# Autodesk Inventor assembly: assembly
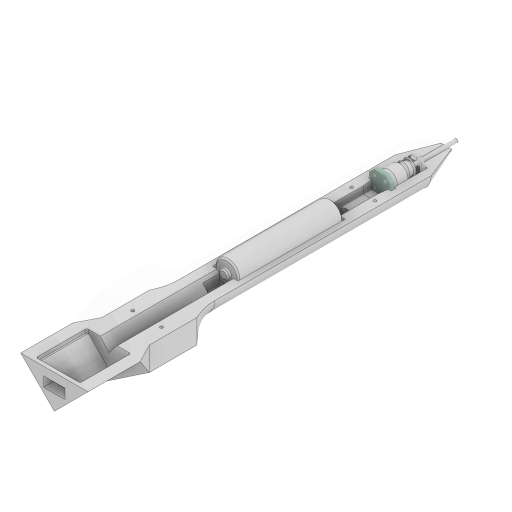
[picture p0: Inventor's stored thumbnail of the model, 512x512]
Saved by Autodesk Inventor 2023 (Build 270158000, 158)
## iProperties
Created: 2023-03-22
Part Number: assembly
Document SubType Name: Assembly
Designer: James
Author: James
## iProperties of the stored document dpoint PCB.ipt
Created: 2023-07-01
Part Number: dpoint PCB
Material: Generic
Document SubType Name: Modeling
Designer: James
Density: 1 g/cm^3
Appearance: Default
Author: James
## iProperties of the stored document COMPOUND.ipt
Created: 2023-07-01
Part Number: COMPOUND
Material: Generic
Document SubType Name: Modeling
Designer: James
Density: 1 g/cm^3
Appearance: Default
Author: James
## iProperties of the stored document ForceSensor(HSFPAR003A).iam
Created: 2023-07-01
Part Number: ForceSensor(HSFPAR003A)
Document SubType Name: Assembly
Designer: James
Author: James
## iProperties of the stored document dpoint.iam
Company: Kicad
Created: 2023-07-02
Part Number: dpoint 1
Description: KiCad electronic assembly
Document SubType Name: Assembly
Designer: James
Authority: Unknown
Sending System: KiCad to STEP converter
Preprocessor: Open CASCADE STEP processor 7.6
Title: dpoint.step
Author: Pcbnew
## Documents named in this file (12)
- C:\Users\James\OneDrive\Documents\Uni\2023_S1\ENG401_honours\inventor\assembly.iam
- C:\Users\James\OneDrive\Documents\Uni\2023_S1\ENG401_honours\inventor\stlyus_body.ipt
- C:\Users\James\OneDrive\Documents\Uni\2023_S1\ENG401_honours\inventor\stylus_nib.ipt
- C:\Users\James\OneDrive\Documents\Uni\2023_S1\ENG401_honours\inventor\seed_arduino.ipt
- C:\Users\James\OneDrive\Documents\Uni\2023_S1\ENG401_honours\inventor\stylus_nib_base.ipt
- C:\Users\James\OneDrive\Documents\Uni\2023_S1\ENG401_honours\inventor\Compress Spring11.ipt
- **C:\Users\James\OneDrive\Documents\Uni\2023_S1\ENG401_honours\inventor\assembly.iam*LocalDocs*xAaaaqsaaAaaaaaaaAaaaqwdiHg*dpoint.iam
- C:\Users\James\OneDrive\Documents\Uni\2023_S1\ENG401_honours\inventor\batt_10440.ipt
- **C:\Users\James\OneDrive\Documents\Uni\2023_S1\ENG401_honours\inventor\assembly.iam*LocalDocs*xAaaaq4daAaaaaaaaAaaaqsjtPd*dpoint PCB.ipt
- **C:\Users\James\OneDrive\Documents\Uni\2023_S1\ENG401_honours\inventor\assembly.iam*LocalDocs*xAaaaavbaAaaaaaaaAaaaaf43Ph*COMPOUND.ipt
- **C:\Users\James\OneDrive\Documents\Uni\2023_S1\ENG401_honours\inventor\assembly.iam*LocalDocs*xAaaaqdbaAaaaaaaaAaaaqo3uAf*ForceSensor(HSFPAR003A).iam
- C:\Users\James\OneDrive\Documents\Uni\2023_S1\ENG401_honours\inventor\dpoint.step
## Components (8 placed, 7 different names)
1. stlyus_body:1 — Mate:1, Flush:1, Mate:2, Mate:3, Flush:2, Flush:7, Flush:3, Mate:8, Mate:9, Insert:2
2. stlyus_body:2 — Mate:1, Flush:1, Mate:2, Mate:7, Flush:8
3. stylus_nib:1 — Mate:3, Insert:1
4. seed_arduino:1 — Flush:2, Flush:7, Flush:3
5. stylus_nib_base:1 — Insert:1, Mate:10
6. Compress Spring1:1 — Mate:7, Mate:8
7. dpoint:1 [sub-assembly] — Mate:9, Mate:10, Mate:11
8. batt_10440:1 — Insert:2
## Relationships (15: Mate 8, Flush 5, Insert 2)
- Mate:1: stlyus_body:1 ↔ stlyus_body:2
- Flush:1: stlyus_body:1 ↔ stlyus_body:2
- Mate:2: stlyus_body:1 ↔ stlyus_body:2
- Mate:3: stlyus_body:1 ↔ stylus_nib:1
- Flush:2: stlyus_body:1 ↔ seed_arduino:1
- Flush:7: stlyus_body:1 ↔ seed_arduino:1
- Flush:3: stlyus_body:1 ↔ seed_arduino:1
- Insert:1: stylus_nib:1 ↔ stylus_nib_base:1
- Mate:7: stlyus_body:2 ↔ Compress Spring1:1
- Mate:8 (0.25 mm): stlyus_body:1 ↔ Compress Spring1:1
- Flush:8 (-5 mm): stlyus_body:2
- Mate:9: stlyus_body:1 ↔ dpoint:1
- Mate:10 (0.5 mm): stylus_nib_base:1 ↔ dpoint:1
- Mate:11: dpoint:1
- Insert:2 (0.5 mm): stlyus_body:1 ↔ batt_10440:1
